# Autodesk Inventor assembly: VersaBlock Assembly
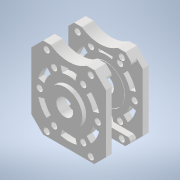
[picture p0: Inventor's stored thumbnail of the model, 180x180]
Saved by Autodesk Inventor 2020 (Build 240168000, 168)
## iProperties
Created: 2020-01-16
Part Number: VersaBlock Assembly
Document SubType Name: Assembly
Designer: aidan
Author: aidan
## Documents named in this file (3)
- C:\Users\aidan\Desktop\T3 Robotics\VersaBlock Assembly.iam
- C:\Users\aidan\Desktop\T3 Robotics\Versa Chassis Bearing Block.ipt
- C:\Users\aidan\Desktop\T3 Robotics\Bearing for THUNDER.ipt
## Components (4 placed, 2 different names)
1. Versa Chassis Bearing Block:1 — Flush:1, Flush:2, Mate:1, Mate:3, Flush:4
2. Versa Chassis Bearing Block:2 — Flush:1, Flush:2, Mate:1, Flush:3, Mate:2
3. Bearing for THUNDER:1 — Mate:3, Flush:4
4. Bearing for THUNDER:2 — Flush:3, Mate:2
## Relationships (7: Flush 4, Mate 3)
- Flush:1: Versa Chassis Bearing Block:1 ↔ Versa Chassis Bearing Block:2
- Flush:2: Versa Chassis Bearing Block:1 ↔ Versa Chassis Bearing Block:2
- Mate:1 (25.4 mm): Versa Chassis Bearing Block:1 ↔ Versa Chassis Bearing Block:2
- Flush:3: Versa Chassis Bearing Block:2 ↔ Bearing for THUNDER:2
- Mate:2: Versa Chassis Bearing Block:2 ↔ Bearing for THUNDER:2
- Mate:3: Versa Chassis Bearing Block:1 ↔ Bearing for THUNDER:1
- Flush:4: Versa Chassis Bearing Block:1 ↔ Bearing for THUNDER:1
